# Autodesk Inventor assembly: 13 in^3 drivetrain
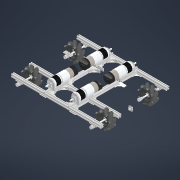
[picture p0: Inventor's stored thumbnail of the model, 180x180]
Saved by Autodesk Inventor 2022 (Build 260153000, 153)
## iProperties
Created: 2021-10-01
Part Number: 13 in^3 drivetrain
Document SubType Name: Assembly
Designer: izack
Author: izack
## Documents named in this file (17)
- C:\Users\elysi\OneDrive\Desktop\ComputerAidedDesign\2021-22\FTC\#12456 Big Red\Proof of Concept\13 in^3 drivetrain.iam
- C:\Users\elysi\OneDrive\Desktop\ComputerAidedDesign\2021-22\FTC\#13822 Robovikes\Proof of Concept\15mm Extrusion - 330.2mm - 90° Ends.ipt
- C:\Users\elysi\OneDrive\Desktop\ComputerAidedDesign\2021-22\FTC\#13822 Robovikes\Proof of Concept\13in^3 drivetrain parts\15mm Bearing Pillow Block - 8 Pack.ipt
- C:\Users\elysi\OneDrive\Desktop\ComputerAidedDesign\2021-22\FTC\#13822 Robovikes\Proof of Concept\13in^3 drivetrain parts\Through Bore Bearing - Long - 12 Pack.ipt
- C:\Users\elysi\OneDrive\Desktop\ComputerAidedDesign\2021-22\FTC\#13822 Robovikes\Proof of Concept\13in^3 drivetrain parts\5mm x 100mm Hex Shaft - 4 Pack.ipt
- C:\Users\elysi\OneDrive\Desktop\ComputerAidedDesign\2021-22\FTC\#13822 Robovikes\Proof of Concept\13in^3 drivetrain parts\Shaft Collars - 10 Pack.ipt
- C:\Users\elysi\OneDrive\Desktop\ComputerAidedDesign\2021-22\FTC\#13822 Robovikes\Proof of Concept\13in^3 drivetrain parts\75mm Mecanum Wheel Set.iam
- C:\Users\elysi\OneDrive\Desktop\ComputerAidedDesign\2021-22\FTC\#13822 Robovikes\Proof of Concept\13in^3 drivetrain parts\15mm Extrusion - 2.5in - 90° Ends.ipt
- C:\Users\elysi\OneDrive\Desktop\ComputerAidedDesign\2021-22\FTC\#13822 Robovikes\Proof of Concept\13in^3 drivetrain parts\15mm Extrusion - 5.637 in - 90° Ends.ipt
- C:\Users\elysi\OneDrive\Desktop\ComputerAidedDesign\2021-22\FTC\#13822 Robovikes\Proof of Concept\26 Tooth #25 Sprocket - 4 Pack.ipt
- C:\Users\elysi\OneDrive\Desktop\ComputerAidedDesign\2021-22\FTC\#13822 Robovikes\Proof of Concept\13in^3 drivetrain parts\10 Tooth #25 D-Shaft Sprocket - 4 Pack.ipt
- C:\Users\elysi\OneDrive\Desktop\ComputerAidedDesign\2021-22\FTC\#13822 Robovikes\Proof of Concept\13in^3 drivetrain parts\15mm Plastic Inside Corner Bracket - 8 Pack.ipt
- C:\Users\elysi\OneDrive\Desktop\ComputerAidedDesign\2021-22\FTC\Parts\Custom Parts\NeveRest 20 Orbital Mount.ipt
- C:\Users\elysi\OneDrive\Desktop\ComputerAidedDesign\2021-22\FTC\Parts\AndyMark\am-3637 NeveRest 20 Orbital Gearmotor.iam
- C:\Users\elysi\OneDrive\Desktop\ComputerAidedDesign\2021-22\FTC\Parts\REV Parts\15mm Metal 90 Degree Bracket V2 - 8 Pack.ipt
- C:\Users\elysi\OneDrive\Desktop\ComputerAidedDesign\2021-22\FTC\Parts\REV Parts\10 Tooth #25 Sprocket - 4 Pack.ipt
- C:\Users\elysi\OneDrive\Desktop\ComputerAidedDesign\2021-22\FTC\Parts\REV Parts\3mm Spacer - 16 Pack.ipt
## Components (82 placed, 16 different names)
1. 15mm Extrusion - 330.2mm - 90° Ends:1 — Flush:5, Mate:6, Flush:7, Flush:8, Flush:15, Mate:8, Mate:12, Mate:16, Mate:25, Mate:68, Mate:69, Mate:131, Mate:134, Mate:24, Flush:50, Flush:51, Mate:164, Mate:166, Flush:61, Flush:64
2. 15mm Extrusion - 330.2mm - 90° Ends:4 — Mate:6, Flush:7, Flush:9, Flush:14, Mate:9, Mate:13, Mate:17, Mate:62, Mate:63, Flush:22, Flush:23, Mate:70, Mate:71, Flush:24, Flush:25, Flush:33, Mate:116, Mate:120, Mate:130, Mate:136, Mate:163, Mate:165, Flush:62, Flush:63
3. 15mm Extrusion - 330.2mm - 90° Ends:5 — Mate:4, Flush:6, Flush:11, Flush:12, Mate:10, Mate:14, Mate:18, Mate:23, Mate:64, Mate:65, Mate:66, Mate:67, Flush:20, Flush:21, Mate:89, Flush:40, Mate:112, Mate:117, Mate:122, Mate:128, Mate:161, Flush:57, Mate:162, Flush:59
4. 15mm Extrusion - 330.2mm - 90° Ends:6 — Flush:5, Mate:4, Flush:6, Flush:13, Mate:11, Flush:10, Mate:15, Mate:19, Mate:22, Mate:123, Mate:126, Mate:140, Mate:141, Flush:48, Flush:49, Flush:54, Mate:159, Flush:56
5. 15mm Bearing Pillow Block - 8 Pack:1 — Flush:9, Mate:9, Mate:17, Rotational:2
6. 15mm Bearing Pillow Block - 8 Pack:2 — Flush:8, Mate:8, Mate:16, Rotational:1, Mate:100
7. 15mm Bearing Pillow Block - 8 Pack:3 — Flush:11, Mate:10, Mate:18, Rotational:3
8. 15mm Bearing Pillow Block - 8 Pack:4 — Flush:10, Mate:11, Mate:19, Rotational:4, Mate:94
9. 15mm Bearing Pillow Block - 8 Pack:5 — Flush:13, Mate:15, Rotational:5, Mate:22, Mate:97
10. 15mm Bearing Pillow Block - 8 Pack:6 — Flush:12, Mate:14, Rigid:2, Mate:23
11. 15mm Bearing Pillow Block - 8 Pack:7 — Flush:14, Mate:13, Rigid:1, Mate:24
12. 15mm Bearing Pillow Block - 8 Pack:8 — Flush:15, Mate:12, Rotational:6, Mate:25, Mate:103
13. Through Bore Bearing - Long - 12 Pack:1 — Rotational:1, Mate:26, Mate:44, Mate:45
14. Through Bore Bearing - Long - 12 Pack:2 — Rotational:3, Mate:27, Mate:28, Mate:29, Mate:46, Mate:47
15. Through Bore Bearing - Long - 12 Pack:3 — Rigid:1, Mate:34, Mate:35, Mate:40, Mate:41
16. Through Bore Bearing - Long - 12 Pack:4 — Rotational:6, Mate:36, Mate:37, Mate:38, Mate:39
17. Through Bore Bearing - Long - 12 Pack:5 — Rigid:2, Mate:33, Mate:42, Mate:43
18. Through Bore Bearing - Long - 12 Pack:6 — Rotational:5, Mate:31, Mate:32, Mate:48, Mate:49
19. Through Bore Bearing - Long - 12 Pack:7 — Rotational:4, Mate:30, Mate:50, Mate:51
20. Through Bore Bearing - Long - 12 Pack:8 — Rotational:2, Mate:20, Mate:21, Mate:52, Mate:53
21. 5mm x 100mm Hex Shaft - 4 Pack:1 — Mate:20, Mate:21, Mate:26, Flush:19, Mate:54, Mate:55, Mate:98, Mate:99
22. 5mm x 100mm Hex Shaft - 4 Pack:2 — Mate:27, Mate:28, Mate:29, Mate:30, Flush:18, Mate:60, Mate:61, Mate:90, Mate:91, Mate:92, Mate:93
23. 5mm x 100mm Hex Shaft - 4 Pack:3 — Mate:31, Mate:32, Mate:33, Flush:17, Mate:58, Mate:59, Mate:95, Mate:96, Mate:168, Mate:170, Mate:171
24. 5mm x 100mm Hex Shaft - 4 Pack:4 — Mate:34, Mate:35, Mate:36, Mate:37, Flush:16, Mate:56, Mate:57, Mate:101, Mate:102
25. Shaft Collars - 10 Pack:1 — Mate:50, Mate:51, Flush:18
26. Shaft Collars - 10 Pack:2 — Mate:52, Mate:53
27. Shaft Collars - 10 Pack:3 — Mate:38, Mate:39, Flush:16
28. Shaft Collars - 10 Pack:4 — Mate:40, Mate:41
29. Shaft Collars - 10 Pack:5 — Mate:48, Mate:49, Flush:17
30. Shaft Collars - 10 Pack:6 — Mate:46, Mate:47
31. Shaft Collars - 10 Pack:7 — Mate:44, Mate:45, Flush:19
32. Shaft Collars - 10 Pack:8 — Mate:42, Mate:43
33. 75mm Mecanum Wheel Set:1 [sub-assembly] — Mate:54, Mate:55, Mate:63
34. 75mm Mecanum Wheel Set:2 [sub-assembly] — Mate:60, Mate:61, Mate:65
35. 75mm Mecanum Wheel Set:3 [sub-assembly] — Mate:58, Mate:59, Mate:64, Mate:167
36. 75mm Mecanum Wheel Set:4 [sub-assembly] — Mate:56, Mate:57, Mate:62
37. 15mm Extrusion - 2.5in - 90° Ends:1 — Mate:66, Flush:21, Flush:27, Flush:42, Flush:43, Mate:125, Mate:127, Mate:160
38. 15mm Extrusion - 2.5in - 90° Ends:2 — Mate:67, Flush:20, Flush:28, Flush:41, Mate:121, Mate:124, Flush:55
39. 15mm Extrusion - 2.5in - 90° Ends:3 — Mate:68, Flush:22, Flush:26, Mate:129, Mate:132, Mate:139, Flush:67
40. 15mm Extrusion - 2.5in - 90° Ends:4 — Mate:69, Flush:23, Flush:29, Flush:33, Mate:133, Mate:135, Mate:138, Flush:66
41. 15mm Extrusion - 5.637 in - 90° Ends:1 — Mate:70, Flush:24, Flush:26, Flush:27, Mate:89, Flush:42, Flush:43, Mate:113, Mate:114, Mate:115, Mate:137, Flush:60, Flush:68
42. 15mm Extrusion - 5.637 in - 90° Ends:2 — Mate:71, Flush:25, Flush:28, Flush:29, Flush:40, Flush:41, Mate:118, Mate:119, Mate:137, Flush:58, Flush:65
43. 26 Tooth #25 Sprocket - 4 Pack:1 — Mate:90, Mate:91, Mate:92, Mate:93, Mate:94, Flush:45
44. 26 Tooth #25 Sprocket - 4 Pack:2 — Mate:95, Mate:96, Mate:97, Flush:46
45. 26 Tooth #25 Sprocket - 4 Pack:3 — Mate:98, Mate:99, Mate:100, Flush:44
46. 26 Tooth #25 Sprocket - 4 Pack:4 — Mate:101, Mate:102, Mate:103, Flush:47
47. 10 Tooth #25 D-Shaft Sprocket - 4 Pack:1 — Flush:44, Mate:156
48. 10 Tooth #25 D-Shaft Sprocket - 4 Pack:2 — Flush:45, Mate:157
49. 10 Tooth #25 D-Shaft Sprocket - 4 Pack:3 — Flush:47, Mate:155
50. 10 Tooth #25 D-Shaft Sprocket - 4 Pack:4 — Flush:46, Mate:158
51. 15mm Plastic Inside Corner Bracket - 8 Pack:1 — Mate:117, Mate:118
52. 15mm Plastic Inside Corner Bracket - 8 Pack:2 — Mate:131, Mate:132
53. 15mm Plastic Inside Corner Bracket - 8 Pack:3 — Mate:112, Mate:113, Mate:114
54. 15mm Plastic Inside Corner Bracket - 8 Pack:4 — Mate:115, Mate:116
55. 15mm Plastic Inside Corner Bracket - 8 Pack:5 — Mate:127, Mate:128
56. 15mm Plastic Inside Corner Bracket - 8 Pack:6 — Mate:129, Mate:130
57. 15mm Plastic Inside Corner Bracket - 8 Pack:7 — Mate:121, Mate:122
58. 15mm Plastic Inside Corner Bracket - 8 Pack:8 — Mate:119, Mate:120
59. 15mm Plastic Inside Corner Bracket - 8 Pack:9 — Mate:125, Mate:126
60. 15mm Plastic Inside Corner Bracket - 8 Pack:10 — Mate:123, Mate:124
61. 15mm Plastic Inside Corner Bracket - 8 Pack:11 — Mate:133, Mate:134
62. 15mm Plastic Inside Corner Bracket - 8 Pack:12 — Mate:135, Mate:136
63. NeveRest 20 Orbital Mount:1 — Mate:140, Flush:49, Mate:146, Mate:148, Mate:152, Flush:53
64. NeveRest 20 Orbital Mount:2 — Mate:141, Flush:48, Mate:147, Mate:153, Mate:154, Flush:52
65. NeveRest 20 Orbital Mount:3 — Mate:139, Flush:50, Mate:145, Mate:149, Mate:151, Flush:53
66. NeveRest 20 Orbital Mount:4 — Mate:138, Flush:51, Mate:142, Mate:143, Mate:144, Flush:52
67. am-3637 NeveRest 20 Orbital Gearmotor:1 [sub-assembly] — Mate:145, Mate:149, Mate:151, Mate:155
68. am-3637 NeveRest 20 Orbital Gearmotor:2 [sub-assembly] — Mate:146, Mate:148, Mate:152, Mate:158
69. am-3637 NeveRest 20 Orbital Gearmotor:3 [sub-assembly] — Mate:147, Mate:153, Mate:154, Mate:157
70. am-3637 NeveRest 20 Orbital Gearmotor:4 [sub-assembly] — Mate:142, Mate:143, Mate:144, Mate:156
71. 15mm Metal 90 Degree Bracket V2 - 8 Pack:1 — Flush:54, Mate:159, Flush:55
72. 15mm Metal 90 Degree Bracket V2 - 8 Pack:2 — Mate:162, Flush:59, Flush:60
73. 15mm Metal 90 Degree Bracket V2 - 8 Pack:3 — Flush:56, Mate:160
74. 15mm Metal 90 Degree Bracket V2 - 8 Pack:4 — Mate:161, Flush:57, Flush:58
75. 15mm Metal 90 Degree Bracket V2 - 8 Pack:5 — Mate:163, Flush:63, Flush:65
76. 15mm Metal 90 Degree Bracket V2 - 8 Pack:6 — Mate:165, Flush:62, Flush:68
77. 15mm Metal 90 Degree Bracket V2 - 8 Pack:7 — Mate:164, Flush:64, Flush:66
78. 15mm Metal 90 Degree Bracket V2 - 8 Pack:8 — Mate:166, Flush:61, Flush:67
79. 10 Tooth #25 Sprocket - 4 Pack:1 — Mate:167, Mate:168, Mate:169
80. 10 Tooth #25 Sprocket - 4 Pack:2 — Mate:169, Mate:170, Mate:172
81. 3mm Spacer - 16 Pack:1 — Mate:171, Mate:172
82. 10 Tooth #25 Sprocket - 4 Pack:3
## Relationships (204: Mate 141, Flush 55, RevoluteJoint 6, WeldJoint 2)
- Flush:5: 15mm Extrusion - 330.2mm - 90° Ends:1 ↔ 15mm Extrusion - 330.2mm - 90° Ends:6
- Mate:4 (68.072 mm): 15mm Extrusion - 330.2mm - 90° Ends:5 ↔ 15mm Extrusion - 330.2mm - 90° Ends:6
- Flush:6: 15mm Extrusion - 330.2mm - 90° Ends:5 ↔ 15mm Extrusion - 330.2mm - 90° Ends:6
- Mate:6 (68.072 mm): 15mm Extrusion - 330.2mm - 90° Ends:1 ↔ 15mm Extrusion - 330.2mm - 90° Ends:4
- Flush:7: 15mm Extrusion - 330.2mm - 90° Ends:1 ↔ 15mm Extrusion - 330.2mm - 90° Ends:4
- Flush:8: 15mm Extrusion - 330.2mm - 90° Ends:1 ↔ 15mm Bearing Pillow Block - 8 Pack:2
- Flush:9: 15mm Extrusion - 330.2mm - 90° Ends:4 ↔ 15mm Bearing Pillow Block - 8 Pack:1
- Flush:10: 15mm Extrusion - 330.2mm - 90° Ends:6 ↔ 15mm Bearing Pillow Block - 8 Pack:4
- Flush:11: 15mm Extrusion - 330.2mm - 90° Ends:5 ↔ 15mm Bearing Pillow Block - 8 Pack:3
- Flush:12: 15mm Extrusion - 330.2mm - 90° Ends:5 ↔ 15mm Bearing Pillow Block - 8 Pack:6
- Flush:13: 15mm Extrusion - 330.2mm - 90° Ends:6 ↔ 15mm Bearing Pillow Block - 8 Pack:5
- Flush:14: 15mm Extrusion - 330.2mm - 90° Ends:4 ↔ 15mm Bearing Pillow Block - 8 Pack:7
- Flush:15: 15mm Extrusion - 330.2mm - 90° Ends:1 ↔ 15mm Bearing Pillow Block - 8 Pack:8
- Mate:8: 15mm Extrusion - 330.2mm - 90° Ends:1 ↔ 15mm Bearing Pillow Block - 8 Pack:2
- Mate:9: 15mm Extrusion - 330.2mm - 90° Ends:4 ↔ 15mm Bearing Pillow Block - 8 Pack:1
- Mate:10: 15mm Extrusion - 330.2mm - 90° Ends:5 ↔ 15mm Bearing Pillow Block - 8 Pack:3
- Mate:11: 15mm Extrusion - 330.2mm - 90° Ends:6 ↔ 15mm Bearing Pillow Block - 8 Pack:4
- Mate:12: 15mm Extrusion - 330.2mm - 90° Ends:1 ↔ 15mm Bearing Pillow Block - 8 Pack:8
- Mate:13: 15mm Extrusion - 330.2mm - 90° Ends:4 ↔ 15mm Bearing Pillow Block - 8 Pack:7
- Mate:14: 15mm Extrusion - 330.2mm - 90° Ends:5 ↔ 15mm Bearing Pillow Block - 8 Pack:6
- Mate:15: 15mm Extrusion - 330.2mm - 90° Ends:6 ↔ 15mm Bearing Pillow Block - 8 Pack:5
- Mate:16 (-19.05 mm): 15mm Extrusion - 330.2mm - 90° Ends:1 ↔ 15mm Bearing Pillow Block - 8 Pack:2
- Mate:17 (-19.05 mm): 15mm Extrusion - 330.2mm - 90° Ends:4 ↔ 15mm Bearing Pillow Block - 8 Pack:1
- Mate:18 (-19.05 mm): 15mm Extrusion - 330.2mm - 90° Ends:5 ↔ 15mm Bearing Pillow Block - 8 Pack:3
- Mate:19 (-19.05 mm): 15mm Extrusion - 330.2mm - 90° Ends:6 ↔ 15mm Bearing Pillow Block - 8 Pack:4
- Rotational:1 [RevoluteJoint]: 15mm Bearing Pillow Block - 8 Pack:2 ↔ Through Bore Bearing - Long - 12 Pack:1
- Rotational:2 [RevoluteJoint]: 15mm Bearing Pillow Block - 8 Pack:1 ↔ Through Bore Bearing - Long - 12 Pack:8
- Rotational:3 [RevoluteJoint]: 15mm Bearing Pillow Block - 8 Pack:3 ↔ Through Bore Bearing - Long - 12 Pack:2
- Rotational:4 [RevoluteJoint]: 15mm Bearing Pillow Block - 8 Pack:4 ↔ Through Bore Bearing - Long - 12 Pack:7
- Rotational:5 [RevoluteJoint]: 15mm Bearing Pillow Block - 8 Pack:5 ↔ Through Bore Bearing - Long - 12 Pack:6
- Rigid:1 [WeldJoint]: 15mm Bearing Pillow Block - 8 Pack:7 ↔ Through Bore Bearing - Long - 12 Pack:3
- Rigid:2 [WeldJoint]: 15mm Bearing Pillow Block - 8 Pack:6 ↔ Through Bore Bearing - Long - 12 Pack:5
- Rotational:6 [RevoluteJoint]: 15mm Bearing Pillow Block - 8 Pack:8 ↔ Through Bore Bearing - Long - 12 Pack:4
- Mate:20: Through Bore Bearing - Long - 12 Pack:8 ↔ 5mm x 100mm Hex Shaft - 4 Pack:1
- Mate:21: Through Bore Bearing - Long - 12 Pack:8 ↔ 5mm x 100mm Hex Shaft - 4 Pack:1
- Mate:22 (-19.05 mm): 15mm Extrusion - 330.2mm - 90° Ends:6 ↔ 15mm Bearing Pillow Block - 8 Pack:5
- Mate:23 (-19.05 mm): 15mm Extrusion - 330.2mm - 90° Ends:5 ↔ 15mm Bearing Pillow Block - 8 Pack:6
- Mate:24 (-19.05 mm): 15mm Extrusion - 330.2mm - 90° Ends:1 ↔ 15mm Bearing Pillow Block - 8 Pack:7
- Mate:25 (-19.05 mm): 15mm Extrusion - 330.2mm - 90° Ends:1 ↔ 15mm Bearing Pillow Block - 8 Pack:8
- Mate:26: Through Bore Bearing - Long - 12 Pack:1 ↔ 5mm x 100mm Hex Shaft - 4 Pack:1
- Mate:27: Through Bore Bearing - Long - 12 Pack:2 ↔ 5mm x 100mm Hex Shaft - 4 Pack:2
- Mate:28: Through Bore Bearing - Long - 12 Pack:2 ↔ 5mm x 100mm Hex Shaft - 4 Pack:2
- Mate:29: Through Bore Bearing - Long - 12 Pack:2 ↔ 5mm x 100mm Hex Shaft - 4 Pack:2
- Mate:30: Through Bore Bearing - Long - 12 Pack:7 ↔ 5mm x 100mm Hex Shaft - 4 Pack:2
- Mate:31: Through Bore Bearing - Long - 12 Pack:6 ↔ 5mm x 100mm Hex Shaft - 4 Pack:3
- Mate:32: Through Bore Bearing - Long - 12 Pack:6 ↔ 5mm x 100mm Hex Shaft - 4 Pack:3
- Mate:33: Through Bore Bearing - Long - 12 Pack:5 ↔ 5mm x 100mm Hex Shaft - 4 Pack:3
- Mate:34: Through Bore Bearing - Long - 12 Pack:3 ↔ 5mm x 100mm Hex Shaft - 4 Pack:4
- Mate:35: Through Bore Bearing - Long - 12 Pack:3 ↔ 5mm x 100mm Hex Shaft - 4 Pack:4
- Mate:36: Through Bore Bearing - Long - 12 Pack:4 ↔ 5mm x 100mm Hex Shaft - 4 Pack:4
- Mate:37: Through Bore Bearing - Long - 12 Pack:4 ↔ 5mm x 100mm Hex Shaft - 4 Pack:4
- Mate:38: Through Bore Bearing - Long - 12 Pack:4 ↔ Shaft Collars - 10 Pack:3
- Mate:39: Through Bore Bearing - Long - 12 Pack:4 ↔ Shaft Collars - 10 Pack:3
- Flush:16: 5mm x 100mm Hex Shaft - 4 Pack:4 ↔ Shaft Collars - 10 Pack:3
- Mate:40: Through Bore Bearing - Long - 12 Pack:3 ↔ Shaft Collars - 10 Pack:4
- Mate:41: Through Bore Bearing - Long - 12 Pack:3 ↔ Shaft Collars - 10 Pack:4
- Mate:42: Through Bore Bearing - Long - 12 Pack:5 ↔ Shaft Collars - 10 Pack:8
- Mate:43: Through Bore Bearing - Long - 12 Pack:5 ↔ Shaft Collars - 10 Pack:8
- Mate:44: Through Bore Bearing - Long - 12 Pack:1 ↔ Shaft Collars - 10 Pack:7
- Mate:45: Through Bore Bearing - Long - 12 Pack:1 ↔ Shaft Collars - 10 Pack:7
- Mate:46: Through Bore Bearing - Long - 12 Pack:2 ↔ Shaft Collars - 10 Pack:6
- Mate:47: Through Bore Bearing - Long - 12 Pack:2 ↔ Shaft Collars - 10 Pack:6
- Mate:48: Through Bore Bearing - Long - 12 Pack:6 ↔ Shaft Collars - 10 Pack:5
- Mate:49: Through Bore Bearing - Long - 12 Pack:6 ↔ Shaft Collars - 10 Pack:5
- Mate:50: Through Bore Bearing - Long - 12 Pack:7 ↔ Shaft Collars - 10 Pack:1
- Mate:51: Through Bore Bearing - Long - 12 Pack:7 ↔ Shaft Collars - 10 Pack:1
- Mate:52: Through Bore Bearing - Long - 12 Pack:8 ↔ Shaft Collars - 10 Pack:2
- Mate:53: Through Bore Bearing - Long - 12 Pack:8 ↔ Shaft Collars - 10 Pack:2
- Flush:17: 5mm x 100mm Hex Shaft - 4 Pack:3 ↔ Shaft Collars - 10 Pack:5
- Flush:18: 5mm x 100mm Hex Shaft - 4 Pack:2 ↔ Shaft Collars - 10 Pack:1
- Flush:19: 5mm x 100mm Hex Shaft - 4 Pack:1 ↔ Shaft Collars - 10 Pack:7
- Mate:54: 5mm x 100mm Hex Shaft - 4 Pack:1 ↔ 75mm Mecanum Wheel Set:1
- Mate:55: 5mm x 100mm Hex Shaft - 4 Pack:1 ↔ 75mm Mecanum Wheel Set:1
- Mate:56: 5mm x 100mm Hex Shaft - 4 Pack:4 ↔ 75mm Mecanum Wheel Set:4
- Mate:57: 5mm x 100mm Hex Shaft - 4 Pack:4 ↔ 75mm Mecanum Wheel Set:4
- Mate:58: 5mm x 100mm Hex Shaft - 4 Pack:3 ↔ 75mm Mecanum Wheel Set:3
- Mate:59: 5mm x 100mm Hex Shaft - 4 Pack:3 ↔ 75mm Mecanum Wheel Set:3
- Mate:60: 5mm x 100mm Hex Shaft - 4 Pack:2 ↔ 75mm Mecanum Wheel Set:2
- Mate:61: 5mm x 100mm Hex Shaft - 4 Pack:2 ↔ 75mm Mecanum Wheel Set:2
- Mate:62 (16.51 mm): 15mm Extrusion - 330.2mm - 90° Ends:4 ↔ 75mm Mecanum Wheel Set:4
- Mate:63 (16.51 mm): 15mm Extrusion - 330.2mm - 90° Ends:4 ↔ 75mm Mecanum Wheel Set:1
- Mate:64 (21.082 mm): 15mm Extrusion - 330.2mm - 90° Ends:5 ↔ 75mm Mecanum Wheel Set:3
- Mate:65 (21.082 mm): 15mm Extrusion - 330.2mm - 90° Ends:5 ↔ 75mm Mecanum Wheel Set:2
- Mate:66: 15mm Extrusion - 330.2mm - 90° Ends:5 ↔ 15mm Extrusion - 2.5in - 90° Ends:1
- Mate:67: 15mm Extrusion - 330.2mm - 90° Ends:5 ↔ 15mm Extrusion - 2.5in - 90° Ends:2
- Flush:20: 15mm Extrusion - 330.2mm - 90° Ends:5 ↔ 15mm Extrusion - 2.5in - 90° Ends:2
- Flush:21: 15mm Extrusion - 330.2mm - 90° Ends:5 ↔ 15mm Extrusion - 2.5in - 90° Ends:1
- Mate:68: 15mm Extrusion - 330.2mm - 90° Ends:1 ↔ 15mm Extrusion - 2.5in - 90° Ends:3
- Mate:69: 15mm Extrusion - 330.2mm - 90° Ends:1 ↔ 15mm Extrusion - 2.5in - 90° Ends:4
- Flush:22: 15mm Extrusion - 330.2mm - 90° Ends:4 ↔ 15mm Extrusion - 2.5in - 90° Ends:3
- Flush:23: 15mm Extrusion - 330.2mm - 90° Ends:4 ↔ 15mm Extrusion - 2.5in - 90° Ends:4
- Mate:70: 15mm Extrusion - 330.2mm - 90° Ends:4 ↔ 15mm Extrusion - 5.637 in - 90° Ends:1
- Mate:71: 15mm Extrusion - 330.2mm - 90° Ends:4 ↔ 15mm Extrusion - 5.637 in - 90° Ends:2
- Flush:24: 15mm Extrusion - 330.2mm - 90° Ends:4 ↔ 15mm Extrusion - 5.637 in - 90° Ends:1
- Flush:25: 15mm Extrusion - 330.2mm - 90° Ends:4 ↔ 15mm Extrusion - 5.637 in - 90° Ends:2
- Flush:26: 15mm Extrusion - 2.5in - 90° Ends:3 ↔ 15mm Extrusion - 5.637 in - 90° Ends:1
- Flush:27: 15mm Extrusion - 2.5in - 90° Ends:1 ↔ 15mm Extrusion - 5.637 in - 90° Ends:1
- Flush:28: 15mm Extrusion - 2.5in - 90° Ends:2 ↔ 15mm Extrusion - 5.637 in - 90° Ends:2
- Flush:29: 15mm Extrusion - 2.5in - 90° Ends:4 ↔ 15mm Extrusion - 5.637 in - 90° Ends:2
- Flush:33 (152.4 mm): 15mm Extrusion - 330.2mm - 90° Ends:4 ↔ 15mm Extrusion - 2.5in - 90° Ends:4
- Mate:89: 15mm Extrusion - 330.2mm - 90° Ends:5 ↔ 15mm Extrusion - 5.637 in - 90° Ends:1
- Flush:40: 15mm Extrusion - 330.2mm - 90° Ends:5 ↔ 15mm Extrusion - 5.637 in - 90° Ends:2
- Flush:41: 15mm Extrusion - 2.5in - 90° Ends:2 ↔ 15mm Extrusion - 5.637 in - 90° Ends:2
- Flush:42: 15mm Extrusion - 2.5in - 90° Ends:1 ↔ 15mm Extrusion - 5.637 in - 90° Ends:1
- Flush:43: 15mm Extrusion - 2.5in - 90° Ends:1 ↔ 15mm Extrusion - 5.637 in - 90° Ends:1
- Mate:90: 5mm x 100mm Hex Shaft - 4 Pack:2 ↔ 26 Tooth #25 Sprocket - 4 Pack:1
- Mate:91: 5mm x 100mm Hex Shaft - 4 Pack:2 ↔ 26 Tooth #25 Sprocket - 4 Pack:1
- Mate:92: 5mm x 100mm Hex Shaft - 4 Pack:2 ↔ 26 Tooth #25 Sprocket - 4 Pack:1
- Mate:93: 5mm x 100mm Hex Shaft - 4 Pack:2 ↔ 26 Tooth #25 Sprocket - 4 Pack:1
- Mate:94 (2.54 mm): 15mm Bearing Pillow Block - 8 Pack:4 ↔ 26 Tooth #25 Sprocket - 4 Pack:1
- Mate:95: 5mm x 100mm Hex Shaft - 4 Pack:3 ↔ 26 Tooth #25 Sprocket - 4 Pack:2
- Mate:96: 5mm x 100mm Hex Shaft - 4 Pack:3 ↔ 26 Tooth #25 Sprocket - 4 Pack:2
- Mate:97 (2.54 mm): 15mm Bearing Pillow Block - 8 Pack:5 ↔ 26 Tooth #25 Sprocket - 4 Pack:2
- Mate:98: 5mm x 100mm Hex Shaft - 4 Pack:1 ↔ 26 Tooth #25 Sprocket - 4 Pack:3
- Mate:99: 5mm x 100mm Hex Shaft - 4 Pack:1 ↔ 26 Tooth #25 Sprocket - 4 Pack:3
- Mate:100 (2.54 mm): 15mm Bearing Pillow Block - 8 Pack:2 ↔ 26 Tooth #25 Sprocket - 4 Pack:3
- Mate:101: 5mm x 100mm Hex Shaft - 4 Pack:4 ↔ 26 Tooth #25 Sprocket - 4 Pack:4
- Mate:102: 5mm x 100mm Hex Shaft - 4 Pack:4 ↔ 26 Tooth #25 Sprocket - 4 Pack:4
- Mate:103 (2.54 mm): 15mm Bearing Pillow Block - 8 Pack:8 ↔ 26 Tooth #25 Sprocket - 4 Pack:4
- Flush:44: 26 Tooth #25 Sprocket - 4 Pack:3 ↔ 10 Tooth #25 D-Shaft Sprocket - 4 Pack:1
- Flush:45: 26 Tooth #25 Sprocket - 4 Pack:1 ↔ 10 Tooth #25 D-Shaft Sprocket - 4 Pack:2
- Flush:46: 26 Tooth #25 Sprocket - 4 Pack:2 ↔ 10 Tooth #25 D-Shaft Sprocket - 4 Pack:4
- Flush:47: 26 Tooth #25 Sprocket - 4 Pack:4 ↔ 10 Tooth #25 D-Shaft Sprocket - 4 Pack:3
- Mate:112: 15mm Extrusion - 330.2mm - 90° Ends:5 ↔ 15mm Plastic Inside Corner Bracket - 8 Pack:3
- Mate:113: 15mm Extrusion - 5.637 in - 90° Ends:1 ↔ 15mm Plastic Inside Corner Bracket - 8 Pack:3
- Mate:114 (0.381 mm): 15mm Extrusion - 5.637 in - 90° Ends:1 ↔ 15mm Plastic Inside Corner Bracket - 8 Pack:3
- Mate:115: 15mm Extrusion - 5.637 in - 90° Ends:1 ↔ 15mm Plastic Inside Corner Bracket - 8 Pack:4
- Mate:116: 15mm Extrusion - 330.2mm - 90° Ends:4 ↔ 15mm Plastic Inside Corner Bracket - 8 Pack:4
- Mate:117: 15mm Extrusion - 330.2mm - 90° Ends:5 ↔ 15mm Plastic Inside Corner Bracket - 8 Pack:1
- Mate:118: 15mm Extrusion - 5.637 in - 90° Ends:2 ↔ 15mm Plastic Inside Corner Bracket - 8 Pack:1
- Mate:119: 15mm Extrusion - 5.637 in - 90° Ends:2 ↔ 15mm Plastic Inside Corner Bracket - 8 Pack:8
- Mate:120: 15mm Extrusion - 330.2mm - 90° Ends:4 ↔ 15mm Plastic Inside Corner Bracket - 8 Pack:8
- Mate:121: 15mm Extrusion - 2.5in - 90° Ends:2 ↔ 15mm Plastic Inside Corner Bracket - 8 Pack:7
- Mate:122: 15mm Extrusion - 330.2mm - 90° Ends:5 ↔ 15mm Plastic Inside Corner Bracket - 8 Pack:7
- Mate:123: 15mm Extrusion - 330.2mm - 90° Ends:6 ↔ 15mm Plastic Inside Corner Bracket - 8 Pack:10
- Mate:124: 15mm Extrusion - 2.5in - 90° Ends:2 ↔ 15mm Plastic Inside Corner Bracket - 8 Pack:10
- Mate:125: 15mm Extrusion - 2.5in - 90° Ends:1 ↔ 15mm Plastic Inside Corner Bracket - 8 Pack:9
- Mate:126: 15mm Extrusion - 330.2mm - 90° Ends:6 ↔ 15mm Plastic Inside Corner Bracket - 8 Pack:9
- Mate:127: 15mm Extrusion - 2.5in - 90° Ends:1 ↔ 15mm Plastic Inside Corner Bracket - 8 Pack:5
- Mate:128: 15mm Extrusion - 330.2mm - 90° Ends:5 ↔ 15mm Plastic Inside Corner Bracket - 8 Pack:5
- Mate:129: 15mm Extrusion - 2.5in - 90° Ends:3 ↔ 15mm Plastic Inside Corner Bracket - 8 Pack:6
- Mate:130: 15mm Extrusion - 330.2mm - 90° Ends:4 ↔ 15mm Plastic Inside Corner Bracket - 8 Pack:6
- Mate:131: 15mm Extrusion - 330.2mm - 90° Ends:1 ↔ 15mm Plastic Inside Corner Bracket - 8 Pack:2
- Mate:132: 15mm Extrusion - 2.5in - 90° Ends:3 ↔ 15mm Plastic Inside Corner Bracket - 8 Pack:2
- Mate:133: 15mm Extrusion - 2.5in - 90° Ends:4 ↔ 15mm Plastic Inside Corner Bracket - 8 Pack:11
- Mate:134: 15mm Extrusion - 330.2mm - 90° Ends:1 ↔ 15mm Plastic Inside Corner Bracket - 8 Pack:11
- Mate:135: 15mm Extrusion - 2.5in - 90° Ends:4 ↔ 15mm Plastic Inside Corner Bracket - 8 Pack:12
- Mate:136: 15mm Extrusion - 330.2mm - 90° Ends:4 ↔ 15mm Plastic Inside Corner Bracket - 8 Pack:12
- Mate:137 (101.6 mm): 15mm Extrusion - 5.637 in - 90° Ends:1 ↔ 15mm Extrusion - 5.637 in - 90° Ends:2
- Mate:138: 15mm Extrusion - 2.5in - 90° Ends:4 ↔ NeveRest 20 Orbital Mount:4
- Mate:139: 15mm Extrusion - 2.5in - 90° Ends:3 ↔ NeveRest 20 Orbital Mount:3
- Mate:140: 15mm Extrusion - 330.2mm - 90° Ends:6 ↔ NeveRest 20 Orbital Mount:1
- Mate:141: 15mm Extrusion - 330.2mm - 90° Ends:6 ↔ NeveRest 20 Orbital Mount:2
- Flush:48: 15mm Extrusion - 330.2mm - 90° Ends:6 ↔ NeveRest 20 Orbital Mount:2
- Flush:49: 15mm Extrusion - 330.2mm - 90° Ends:6 ↔ NeveRest 20 Orbital Mount:1
- Flush:50: 15mm Extrusion - 330.2mm - 90° Ends:1 ↔ NeveRest 20 Orbital Mount:3
- Flush:51: 15mm Extrusion - 330.2mm - 90° Ends:1 ↔ NeveRest 20 Orbital Mount:4
- Mate:142: NeveRest 20 Orbital Mount:4 ↔ am-3637 NeveRest 20 Orbital Gearmotor:4
- Mate:143: NeveRest 20 Orbital Mount:4 ↔ am-3637 NeveRest 20 Orbital Gearmotor:4
- Mate:144: NeveRest 20 Orbital Mount:4 ↔ am-3637 NeveRest 20 Orbital Gearmotor:4
- Mate:145: NeveRest 20 Orbital Mount:3 ↔ am-3637 NeveRest 20 Orbital Gearmotor:1
- Mate:146: NeveRest 20 Orbital Mount:1 ↔ am-3637 NeveRest 20 Orbital Gearmotor:2
- Mate:147: NeveRest 20 Orbital Mount:2 ↔ am-3637 NeveRest 20 Orbital Gearmotor:3
- Mate:148: NeveRest 20 Orbital Mount:1 ↔ am-3637 NeveRest 20 Orbital Gearmotor:2
- Mate:149: NeveRest 20 Orbital Mount:3 ↔ am-3637 NeveRest 20 Orbital Gearmotor:1
- Mate:151: NeveRest 20 Orbital Mount:3 ↔ am-3637 NeveRest 20 Orbital Gearmotor:1
- Mate:152: NeveRest 20 Orbital Mount:1 ↔ am-3637 NeveRest 20 Orbital Gearmotor:2
- Mate:153: NeveRest 20 Orbital Mount:2 ↔ am-3637 NeveRest 20 Orbital Gearmotor:3
- Mate:154: NeveRest 20 Orbital Mount:2 ↔ am-3637 NeveRest 20 Orbital Gearmotor:3
- Mate:155: 10 Tooth #25 D-Shaft Sprocket - 4 Pack:3 ↔ am-3637 NeveRest 20 Orbital Gearmotor:1
- Mate:156: 10 Tooth #25 D-Shaft Sprocket - 4 Pack:1 ↔ am-3637 NeveRest 20 Orbital Gearmotor:4
- Flush:52: NeveRest 20 Orbital Mount:2 ↔ NeveRest 20 Orbital Mount:4
- Flush:53: NeveRest 20 Orbital Mount:1 ↔ NeveRest 20 Orbital Mount:3
- Mate:157: 10 Tooth #25 D-Shaft Sprocket - 4 Pack:2 ↔ am-3637 NeveRest 20 Orbital Gearmotor:3
- Mate:158: 10 Tooth #25 D-Shaft Sprocket - 4 Pack:4 ↔ am-3637 NeveRest 20 Orbital Gearmotor:2
- Flush:54: 15mm Extrusion - 330.2mm - 90° Ends:6 ↔ 15mm Metal 90 Degree Bracket V2 - 8 Pack:1
- Mate:159: 15mm Extrusion - 330.2mm - 90° Ends:6 ↔ 15mm Metal 90 Degree Bracket V2 - 8 Pack:1
- Flush:55: 15mm Extrusion - 2.5in - 90° Ends:2 ↔ 15mm Metal 90 Degree Bracket V2 - 8 Pack:1
- Flush:56: 15mm Extrusion - 330.2mm - 90° Ends:6 ↔ 15mm Metal 90 Degree Bracket V2 - 8 Pack:3
- Mate:160: 15mm Extrusion - 2.5in - 90° Ends:1 ↔ 15mm Metal 90 Degree Bracket V2 - 8 Pack:3
- Mate:161: 15mm Extrusion - 330.2mm - 90° Ends:5 ↔ 15mm Metal 90 Degree Bracket V2 - 8 Pack:4
- Flush:57: 15mm Extrusion - 330.2mm - 90° Ends:5 ↔ 15mm Metal 90 Degree Bracket V2 - 8 Pack:4
- Flush:58: 15mm Extrusion - 5.637 in - 90° Ends:2 ↔ 15mm Metal 90 Degree Bracket V2 - 8 Pack:4
- Mate:162: 15mm Extrusion - 330.2mm - 90° Ends:5 ↔ 15mm Metal 90 Degree Bracket V2 - 8 Pack:2
- Flush:59: 15mm Extrusion - 330.2mm - 90° Ends:5 ↔ 15mm Metal 90 Degree Bracket V2 - 8 Pack:2
- Flush:60: 15mm Extrusion - 5.637 in - 90° Ends:1 ↔ 15mm Metal 90 Degree Bracket V2 - 8 Pack:2
- Mate:163: 15mm Extrusion - 330.2mm - 90° Ends:4 ↔ 15mm Metal 90 Degree Bracket V2 - 8 Pack:5
- Mate:164: 15mm Extrusion - 330.2mm - 90° Ends:1 ↔ 15mm Metal 90 Degree Bracket V2 - 8 Pack:7
- Mate:165: 15mm Extrusion - 330.2mm - 90° Ends:4 ↔ 15mm Metal 90 Degree Bracket V2 - 8 Pack:6
- Mate:166: 15mm Extrusion - 330.2mm - 90° Ends:1 ↔ 15mm Metal 90 Degree Bracket V2 - 8 Pack:8
- Flush:61: 15mm Extrusion - 330.2mm - 90° Ends:1 ↔ 15mm Metal 90 Degree Bracket V2 - 8 Pack:8
- Flush:62: 15mm Extrusion - 330.2mm - 90° Ends:4 ↔ 15mm Metal 90 Degree Bracket V2 - 8 Pack:6
- Flush:63: 15mm Extrusion - 330.2mm - 90° Ends:4 ↔ 15mm Metal 90 Degree Bracket V2 - 8 Pack:5
- Flush:64: 15mm Extrusion - 330.2mm - 90° Ends:1 ↔ 15mm Metal 90 Degree Bracket V2 - 8 Pack:7
- Flush:65: 15mm Extrusion - 5.637 in - 90° Ends:2 ↔ 15mm Metal 90 Degree Bracket V2 - 8 Pack:5
- Flush:66: 15mm Extrusion - 2.5in - 90° Ends:4 ↔ 15mm Metal 90 Degree Bracket V2 - 8 Pack:7
- Flush:67: 15mm Extrusion - 2.5in - 90° Ends:3 ↔ 15mm Metal 90 Degree Bracket V2 - 8 Pack:8
- Flush:68: 15mm Extrusion - 5.637 in - 90° Ends:1 ↔ 15mm Metal 90 Degree Bracket V2 - 8 Pack:6
- Mate:167: 75mm Mecanum Wheel Set:3 ↔ 10 Tooth #25 Sprocket - 4 Pack:1
- Mate:168: 5mm x 100mm Hex Shaft - 4 Pack:3 ↔ 10 Tooth #25 Sprocket - 4 Pack:1
- Mate:169: 10 Tooth #25 Sprocket - 4 Pack:1 ↔ 10 Tooth #25 Sprocket - 4 Pack:2
- Mate:170: 5mm x 100mm Hex Shaft - 4 Pack:3 ↔ 10 Tooth #25 Sprocket - 4 Pack:2
- Mate:171: 5mm x 100mm Hex Shaft - 4 Pack:3 ↔ 3mm Spacer - 16 Pack:1
- Mate:172: 10 Tooth #25 Sprocket - 4 Pack:2 ↔ 3mm Spacer - 16 Pack:1
